# Autodesk Inventor assembly: ASY ANP 1427 FDS way 7
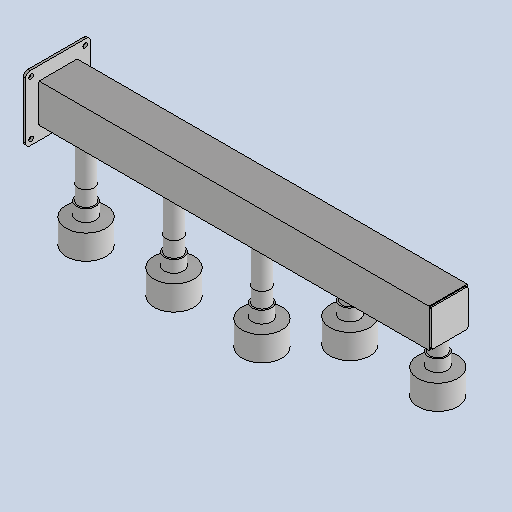
[picture p0: Inventor's stored thumbnail of the model, 512x512]
Saved by Autodesk Inventor 2025 (Build 290162010, 162A)
## iProperties
Created: 2025-07-02
Part Number: ASY ANP 1427 FDS way 7
Document SubType Name: Assembly
Designer: admin
Author: user
## Documents named in this file (7)
- C:\Users\pokla\Documents\Inventor\ANP--Antipayuta\FDS 1400\ASY ANP 1427 FDS way 7.iam
- C:\Users\pokla\Documents\Inventor\ANP--Antipayuta\FDS 1400\ANP 1437 FDS WAY tube7.ipt
- C:\Users\pokla\Documents\Inventor\ANP--Antipayuta\FDS 1400\ANP 1425 FDS Way FLANGE.ipt
- C:\Users\pokla\Documents\Inventor\ANP--Antipayuta\FDS 1400\ANP 1426 FDS way cup.ipt
- C:\Users\pokla\Documents\Inventor\ANP--Antipayuta\FDS 1400\ANP dummy filter element.ipt
- C:\Users\pokla\Documents\Inventor\ANP--Antipayuta\FDS 1400\ANP dummy pipe nippel.ipt
- C:\Users\pokla\Documents\Inventor\ANP--Antipayuta\FDS 1400\ANP 1451 FDS thread  tube10.ipt
## Components (16 placed, 6 different names)
1. TKS 3537 FDS WAY tube7:1 — Rigid:34, Rigid:35, Rigid:36, Rigid:26, Rotational:1, Rotational:2, Rotational:3
2. TKS 3525 FDS Way FLANGE:1 — Rigid:34
3. TKS 3526 FDS way cup:1 — Rigid:35
4. TKS dummy filter element:1 — Rigid:1
5. TKS dummy pipe nippel:1 — Rigid:1, Rotational:1
6. TKS dummy filter element:2 — Rigid:33
7. TKS dummy pipe nippel:2 — Rigid:33, Rigid:36
8. TKS dummy filter element:3 — Rigid:24
9. TKS dummy pipe nippel:3 — Rigid:24, Rigid:25
10. TKS 3551 FDS thread  tube10:1 — Rigid:26, Rigid:25
11. TKS dummy filter element:4
12. TKS dummy pipe nippel:4
13. TKS 3551 FDS thread  tube10:2 — Rotational:2
14. TKS dummy filter element:5
15. TKS dummy pipe nippel:5
16. TKS 3551 FDS thread  tube10:3 — Rotational:3
## Relationships (15: WeldJoint 12, RevoluteJoint 3)
- Rigid:34 [WeldJoint] (2 mm): TKS 3537 FDS WAY tube7:1 ↔ TKS 3525 FDS Way FLANGE:1
- Rigid:35 [WeldJoint]: TKS 3537 FDS WAY tube7:1 ↔ TKS 3526 FDS way cup:1
- Rigid:1 [WeldJoint]: TKS dummy filter element:1 ↔ TKS dummy pipe nippel:1
- Rigid:33 [WeldJoint]: TKS dummy filter element:2 ↔ TKS dummy pipe nippel:2
- Rigid:36 [WeldJoint]: TKS 3537 FDS WAY tube7:1 ↔ TKS dummy pipe nippel:2
- Rigid:24 [WeldJoint]: TKS dummy filter element:3 ↔ TKS dummy pipe nippel:3
- Rigid:26 [WeldJoint]: TKS 3537 FDS WAY tube7:1 ↔ TKS 3551 FDS thread  tube10:1
- Rigid:25 [WeldJoint]: TKS dummy pipe nippel:3 ↔ TKS 3551 FDS thread  tube10:1
- [WeldJoint]: TKS dummy filter element:4 ↔ TKS dummy pipe nippel:4
- [WeldJoint]: TKS dummy pipe nippel:4 ↔ TKS 3551 FDS thread  tube10:2
- [WeldJoint]: TKS dummy filter element:5 ↔ TKS dummy pipe nippel:5
- [WeldJoint]: TKS dummy pipe nippel:5 ↔ TKS 3551 FDS thread  tube10:3
- Rotational:1 [RevoluteJoint]: TKS 3537 FDS WAY tube7:1 ↔ TKS dummy pipe nippel:1
- Rotational:2 [RevoluteJoint]: TKS 3537 FDS WAY tube7:1 ↔ TKS 3551 FDS thread  tube10:2
- Rotational:3 [RevoluteJoint]: TKS 3537 FDS WAY tube7:1 ↔ TKS 3551 FDS thread  tube10:3
## Named parameters: d22_d19 = 0 mm, d23_d21 = 0 mm, d24_d19 = 0 mm, d25_d21 = 0 mm
